# Autodesk Inventor assembly: Assembly1
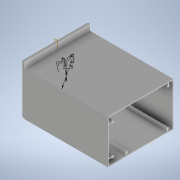
[picture p0: Inventor's stored thumbnail of the model, 180x180]
Saved by Autodesk Inventor 2020.3 (Build 243373000, 373)
## iProperties
Created: 2020-08-10
Part Number: Assembly1
Document SubType Name: Assembly
Designer: joesp
Author: joesp
## Documents named in this file (6)
- C:\Users\joesp\Desktop\fullmotion racing sim\Steering Wheel\chassis\3d models\Assembly1.iam
- C:\Users\joesp\Desktop\fullmotion racing sim\Steering Wheel\chassis\3d models\front plate.ipt
- C:\Users\joesp\Desktop\fullmotion racing sim\Steering Wheel\chassis\3d models\shaft holder.ipt
- C:\Users\joesp\Desktop\fullmotion racing sim\Steering Wheel\chassis\3d models\shaft.ipt
- C:\Users\joesp\Desktop\fullmotion racing sim\Steering Wheel\chassis\3d models\shell.ipt
- C:\Users\joesp\Desktop\fullmotion racing sim\Steering Wheel\chassis\3d models\motor mount.ipt
## Components (5 placed, 5 different names)
1. front plate:1 — Mate:1, Mate:2, Mate:3, Mate:5, Flush:1
2. shaft holder:1 — Mate:3, Mate:4
3. shaft:1 — Mate:1, Mate:2, Mate:4
4. shell:1 — Mate:5, Mate:6, Flush:1
5. motor mount:1 — Mate:6
## Relationships (7: Mate 6, Flush 1)
- Mate:1: front plate:1 ↔ shaft:1
- Mate:2: front plate:1 ↔ shaft:1
- Mate:3: front plate:1 ↔ shaft holder:1
- Mate:4: shaft holder:1 ↔ shaft:1
- Mate:5: front plate:1 ↔ shell:1
- Mate:6: shell:1 ↔ motor mount:1
- Flush:1: front plate:1 ↔ shell:1
